# Autodesk Inventor assembly: 000 Ensamblaje hw_LM - BASIC
(part 2 of 4)
575. UND_0201CR___ _________:138
576. UND_0201CR___ _________:139 — Flush:890
577. UND_0201CR___ _________:140
578. UND_0201CR___ _________:141
579. UND_0201CR___ _________:142
580. UND_0201CR___ _________:143
581. UND_0201CR___ _________:144 — Flush:891, Flush:918
582. UND_0201CR___ _________:145
583. UND_0201CR___ _________:146 — Flush:920
584. UND_0201CR___ _________:147
585. UND_0201CR___ _________:148 — Flush:891
586. UND_0201CR___ _________:149 — Flush:889
587. UND_0201CR___ _________:150
588. UND_0201CR___ _________:151
589. UND_0201CR___ _________:152
590. UND_0201CR___ _________:153
591. UND_0201CR___ _________:154
592. UND_0201CR___ _________:155
593. UND_0201CR___ _________:156
594. UND_0201CR___ _________:157
595. UND_0201CR___ _________:158
596. UND_0201CR___ _________:159 — Flush:918, Flush:919
597. UND_0201CR___ _________:160
598. UND_0201CR___ _________:161
599. UND_0201CR___ _________:162 — Flush:921
600. UND_0201CR___ _________:163
601. UND_0201CR___ _________:164
602. UND_0201CR___ _________:165 — Flush:1036, Flush:1136
603. UND_0201CR___ _________:166
604. UND_0201CR___ _________:167 — Flush:920, Flush:949, Flush:973
605. UND_0201CR___ _________:168 — Flush:919
606. UND_0201CR___ _________:169
607. UND_0201CR___ _________:170 — Flush:953
608. UND_0201CR___ _________:171 — Flush:921, Flush:952
609. UND_0201CR___ _________:172
610. UND_0201CR___ _________:173
611. UND_0201CR___ _________:174
612. UND_0201CR___ _________:175 — Flush:950
613. UND_0201CR___ _________:176 — Flush:948, Flush:949
614. UND_0201CR___ _________:177
615. UND_0201CR___ _________:178 — Flush:952, Flush:974, Flush:998
616. UND_0201CR___ _________:179
617. UND_0201CR___ _________:180 — Flush:951
618. UND_0201CR___ _________:181
619. UND_0201CR___ _________:182 — Flush:953, Flush:976
620. UND_0201CR___ _________:183
621. UND_0201CR___ _________:184
622. UND_0201CR___ _________:185 — Flush:948
623. UND_0201CR___ _________:186
624. UND_0201CR___ _________:187 — Flush:951
625. UND_0201CR___ _________:188
626. UND_0201CR___ _________:189
627. UND_0201CR___ _________:190
628. UND_0201CR___ _________:191 — Flush:950
629. UND_0201CR___ _________:192
630. UND_0201CR___ _________:193 — Flush:973, Flush:976
631. UND_0201CR___ _________:194 — Flush:974
632. UND_0201CR___ _________:195 — Flush:975
633. UND_0201CR___ _________:196
634. UND_0201CR___ _________:197
635. UND_0201CR___ _________:198 — Flush:997
636. UND_0201CR___ _________:199
637. UND_0201CR___ _________:200
638. UND_0201CR___ _________:201 — Flush:996
639. UND_0201CR___ _________:202 — Flush:975
640. UND_0201CR___ _________:203
641. UND_0201CR___ _________:204
642. UND_0201CR___ _________:205
643. UND_0201CR___ _________:206
644. UND_0201CR___ _________:207 — Flush:997
645. UND_0201CR___ _________:208 — Flush:1009
646. UND_0201CR___ _________:209
647. UND_0201CR___ _________:210
648. UND_0201CR___ _________:211
649. UND_0201CR___ _________:212
650. UND_0201CR___ _________:213 — Flush:996
651. UND_0201CR___ _________:214
652. UND_0201CR___ _________:215
653. UND_0201CR___ _________:216
654. UND_0201CR___ _________:217
655. UND_0201CR___ _________:218 — Flush:998
656. UND_0201CR___ _________:219
657. UND_0201CR___ _________:220 — Flush:1008
658. UND_0201CR___ _________:221 — Flush:1008, Flush:1031
659. UND_0201CR___ _________:222
660. UND_0201CR___ _________:223 — Flush:1009
661. UND_0201CR___ _________:224
662. UND_0201CR___ _________:225 — Flush:1032
663. UND_0201CR___ _________:226 — Flush:1029
664. UND_0201CR___ _________:227
665. UND_0201CR___ _________:228
666. UND_0201CR___ _________:229 — Flush:1029, Flush:1069
667. UND_0201CR___ _________:230 — Flush:1033
668. UND_0201CR___ _________:231 — Flush:1034
669. UND_0201CR___ _________:232 — Flush:1030
670. UND_0201CR___ _________:233 — Flush:1031
671. UND_0201CR___ _________:234
672. UND_0201CR___ _________:235
673. UND_0201CR___ _________:236 — Flush:1028, Flush:1036
674. UND_0201CR___ _________:237 — Flush:1033, Flush:1035
675. UND_0201CR___ _________:238 — Flush:1028
676. UND_0201CR___ _________:239
677. UND_0201CR___ _________:240 — Flush:1030, Flush:1034
678. UND_0201CR___ _________:241
679. UND_0201CR___ _________:242 — Flush:1032
680. UND_0201CR___ _________:243
681. UND_0201CR___ _________:244
682. UND_0201CR___ _________:249
683. UND_0201CR___ _________:250
684. UND_0201CR___ _________:251
685. UND_0201CR___ _________:252
686. UND_0201CR___ _________:253
687. UND_0201CR___ _________:257
688. UND_0201CR___ _________:261
689. UND_0201CR___ _________:262
690. UND_0201CR___ _________:266 — Flush:1069
691. UND_0201CR___ _________:267
692. UND_0201CR___ _________:268
693. UND_0201CR___ _________:269 — Flush:1130
694. UND_0201CR___ _________:270 — Flush:1135
695. UND_0201CR___ _________:271 — Flush:1135, Flush:1136
## Relationships (1031: Flush 748, Angle 167, Mate 116)
- Mate:1: hw_LM - PCB:1
- Flush:1: hw_LM - PCB:1
- Flush:2: hw_LM - PCB:1
- Mate:33: hw_LM - PCB:1 ↔ Sen-Z-f:1
- Mate:35: hw_LM - PCB:1 ↔ Sen-XY-f:1
- Flush:16: Sen-XY-f:1 ↔ Sen-XY-f:2
- Mate:60: hw_LM - PCB:1 ↔ MAGI2C:1
- Mate:72: hw_LM - PCB:1 ↔ RES-1.6K_1%_0402:1
- [Flush]: RES-1.6K_1%_0402:9 ↔ RES-1.6K_1%_0402:8
- Flush:59: RES-1.6K_1%_0402:9 ↔ RES-1.6K_1%_0402:8
- Flush:64: RES-1.6K_1%_0402:14 ↔ RES-1.6K_1%_0402:16
- Flush:65: RES-1.6K_1%_0402:14 ↔ RES-1.6K_1%_0402:15
- Flush:66: RES-1.6K_1%_0402:13 ↔ RES-1.6K_1%_0402:15
- [Flush]: RES-1.6K_1%_0402:18 ↔ RES-1.6K_1%_0402:20
- Flush:73: RES-1.6K_1%_0402:16 ↔ RES-1.6K_1%_0402:18
- [Flush]: RES-1.6K_1%_0402:22 ↔ RES-1.6K_1%_0402:25
- [Flush]: RES-1.6K_1%_0402:27 ↔ RES-1.6K_1%_0402:28
- [Flush]: RES-1.6K_1%_0402:27 ↔ RES-1.6K_1%_0402:28
- Flush:85: RES-1.6K_1%_0402:22 ↔ RES-1.6K_1%_0402:27
- Flush:86: RES-1.6K_1%_0402:22 ↔ RES-1.6K_1%_0402:29
- [Flush]: RES-1.6K_1%_0402:34 ↔ RES-1.6K_1%_0402:35
- [Flush]: RES-1.6K_1%_0402:40 ↔ RES-1.6K_1%_0402:42
- Flush:118: RES-1.6K_1%_0402:16 ↔ RES-1.6K_1%_0402:40
- Flush:138: RES-1.6K_1%_0402:44 ↔ RES-1.6K_1%_0402:56
- Mate:84: hw_LM - PCB:1 ↔ RES-1.6K_1%_0402:56
- Flush:146: RES-1.6K_1%_0402:56 ↔ RES-1.6K_1%_0402:58
- Flush:151: RES-1.6K_1%_0402:56 ↔ RES-1.6K_1%_0402:59
- Flush:153: RES-1.6K_1%_0402:50 ↔ RES-1.6K_1%_0402:51
- [Flush]: RES-1.6K_1%_0402:60 ↔ RES-1.6K_1%_0402:62
- Flush:159: RES-1.6K_1%_0402:60 ↔ RES-1.6K_1%_0402:63
- Flush:160: RES-1.6K_1%_0402:61 ↔ RES-1.6K_1%_0402:63
- [Flush]: RES-1.6K_1%_0402:64 ↔ RES-1.6K_1%_0402:66
- [Flush]: RES-1.6K_1%_0402:64 ↔ RES-1.6K_1%_0402:67
- [Flush]: RES-1.6K_1%_0402:65 ↔ RES-1.6K_1%_0402:67
- Flush:164: RES-1.6K_1%_0402:62 ↔ RES-1.6K_1%_0402:65
- [Flush]: RES-1.6K_1%_0402:69 ↔ RES-1.6K_1%_0402:71
- Flush:168: RES-1.6K_1%_0402:62 ↔ RES-1.6K_1%_0402:69
- [Flush]: RES-1.6K_1%_0402:72 ↔ RES-1.6K_1%_0402:73
- [Flush]: RES-1.6K_1%_0402:72 ↔ RES-1.6K_1%_0402:73
- Flush:174: RES-1.6K_1%_0402:72 ↔ RES-1.6K_1%_0402:75
- [Flush]: RES-1.6K_1%_0402:76 ↔ RES-1.6K_1%_0402:77
- [Flush]: RES-1.6K_1%_0402:76 ↔ RES-1.6K_1%_0402:77
- [Flush]: RES-1.6K_1%_0402:78 ↔ RES-1.6K_1%_0402:79
- [Flush]: RES-1.6K_1%_0402:78 ↔ RES-1.6K_1%_0402:79
- [Flush]: RES-1.6K_1%_0402:77 ↔ RES-1.6K_1%_0402:78
- [Flush]: RES-1.6K_1%_0402:76 ↔ RES-1.6K_1%_0402:79
- Flush:182: RES-1.6K_1%_0402:67 ↔ RES-1.6K_1%_0402:79
- Flush:183: RES-1.6K_1%_0402:66 ↔ RES-1.6K_1%_0402:76
- [Flush]: RES-1.6K_1%_0402:80 ↔ RES-1.6K_1%_0402:81
- [Flush]: RES-1.6K_1%_0402:80 ↔ RES-1.6K_1%_0402:81
- Flush:186: RES-1.6K_1%_0402:78 ↔ RES-1.6K_1%_0402:80
- [Flush]: RES-1.6K_1%_0402:84 ↔ RES-1.6K_1%_0402:85
- Flush:192: RES-1.6K_1%_0402:84 ↔ RES-1.6K_1%_0402:85
- Flush:194: RES-1.6K_1%_0402:85 ↔ RES-1.6K_1%_0402:86
- Mate:94: hw_LM - PCB:1 ↔ S32E288ABCAAMJGT:1
- Mate:95: hw_LM - PCB:1 ↔ DP83867ERGZT:1
- Mate:107: hw_LM - PCB:1 ↔ SML-D12V8WT86C:2
- Mate:108: hw_LM - PCB:1 ↔ SML-D12V8WT86C:3
- Mate:109: hw_LM - PCB:1 ↔ SML-D12V8WT86C:4
- Mate:110: hw_LM - PCB:1 ↔ SML-D12V8WT86C:5
- Mate:112: hw_LM - PCB:1 ↔ RES-1.6K_1%_0402:92
- Mate:113: hw_LM - PCB:1 ↔ RES-1.6K_1%_0402:91
- Mate:114: hw_LM - PCB:1 ↔ RES-1.6K_1%_0402:90
- Mate:115: hw_LM - PCB:1 ↔ RES-1.6K_1%_0402:89
- Flush:202: SML-D12V8WT86C:2 ↔ SML-D12V8WT86C:6
- Flush:204: RES-1.6K_1%_0402:89 ↔ RES-1.6K_1%_0402:94
- Flush:205: RES-1.6K_1%_0402:89 ↔ RES-1.6K_1%_0402:90
- Flush:206: RES-1.6K_1%_0402:90 ↔ RES-1.6K_1%_0402:91
- Flush:207: RES-1.6K_1%_0402:91 ↔ RES-1.6K_1%_0402:92
- Mate:116: hw_LM - PCB:1 ↔ SMA6J64CA:1
- Mate:117: hw_LM - PCB:1 ↔ SMA6J64CA:2
- Mate:118: hw_LM - PCB:1 ↔ C1210C472KGRACAUTO:1
- Mate:123: hw_LM - PCB:1 ↔ 1812CAN-113NRC:1
- Mate:124: hw_LM - PCB:1 ↔ TCAN1462VDRBRQ1:5
- Flush:228: C1210C472KGRACAUTO:11 ↔ C1210C472KGRACAUTO:12
- Flush:230: C1210C472KGRACAUTO:11 ↔ C1210C472KGRACAUTO:12
- Flush:232: C1210C472KGRACAUTO:11 ↔ C1210C472KGRACAUTO:12
- [Flush]: RES-1.6K_1%_0402:108 ↔ RES-1.6K_1%_0402:109
- Flush:249: RES-1.6K_1%_0402:107 ↔ RES-1.6K_1%_0402:109
- Flush:251: RES-1.6K_1%_0402:104 ↔ RES-1.6K_1%_0402:109
- Flush:252: RES-1.6K_1%_0402:105 ↔ RES-1.6K_1%_0402:107
- [Flush]: RES-1.6K_1%_0402:114 ↔ RES-1.6K_1%_0402:115
- [Flush]: RES-1.6K_1%_0402:113 ↔ RES-1.6K_1%_0402:115
- [Flush]: RES-1.6K_1%_0402:110 ↔ RES-1.6K_1%_0402:115
- Flush:261: RES-1.6K_1%_0402:105 ↔ RES-1.6K_1%_0402:113
- [Flush]: RES-1.6K_1%_0402:117 ↔ RES-1.6K_1%_0402:118
- [Flush]: RES-1.6K_1%_0402:120 ↔ RES-1.6K_1%_0402:121
- [Flush]: RES-1.6K_1%_0402:118 ↔ RES-1.6K_1%_0402:120
- [Flush]: RES-1.6K_1%_0402:123 ↔ RES-1.6K_1%_0402:124
- Flush:278: RES-1.6K_1%_0402:105 ↔ RES-1.6K_1%_0402:120
- [Flush]: RES-1.6K_1%_0402:129 ↔ RES-1.6K_1%_0402:130
- [Flush]: RES-1.6K_1%_0402:132 ↔ RES-1.6K_1%_0402:133
- [Flush]: RES-1.6K_1%_0402:131 ↔ RES-1.6K_1%_0402:133
- [Flush]: RES-1.6K_1%_0402:130 ↔ RES-1.6K_1%_0402:132
- [Flush]: RES-1.6K_1%_0402:128 ↔ RES-1.6K_1%_0402:133
- [Flush]: RES-1.6K_1%_0402:129 ↔ RES-1.6K_1%_0402:131
- [Flush]: RES-1.6K_1%_0402:135 ↔ RES-1.6K_1%_0402:136
- [Flush]: RES-1.6K_1%_0402:138 ↔ RES-1.6K_1%_0402:139
- [Flush]: RES-1.6K_1%_0402:137 ↔ RES-1.6K_1%_0402:139
- [Flush]: RES-1.6K_1%_0402:136 ↔ RES-1.6K_1%_0402:138
- [Flush]: RES-1.6K_1%_0402:134 ↔ RES-1.6K_1%_0402:139
- [Flush]: RES-1.6K_1%_0402:135 ↔ RES-1.6K_1%_0402:137
- [Flush]: RES-1.6K_1%_0402:131 ↔ RES-1.6K_1%_0402:136
- [Flush]: RES-1.6K_1%_0402:129 ↔ RES-1.6K_1%_0402:137
- [Flush]: RES-1.6K_1%_0402:132 ↔ RES-1.6K_1%_0402:138
- Flush:294: RES-1.6K_1%_0402:134 ↔ RES-1.6K_1%_0402:139
- Flush:295: RES-1.6K_1%_0402:117 ↔ RES-1.6K_1%_0402:139
- Flush:296: RES-1.6K_1%_0402:113 ↔ RES-1.6K_1%_0402:137
- [Flush]: RES-1.6K_1%_0402:140 ↔ RES-1.6K_1%_0402:141
- [Flush]: RES-1.6K_1%_0402:144 ↔ RES-1.6K_1%_0402:145
- [Flush]: RES-1.6K_1%_0402:143 ↔ RES-1.6K_1%_0402:145
- [Flush]: RES-1.6K_1%_0402:142 ↔ RES-1.6K_1%_0402:145
- [Flush]: RES-1.6K_1%_0402:148 ↔ RES-1.6K_1%_0402:149
- [Flush]: RES-1.6K_1%_0402:147 ↔ RES-1.6K_1%_0402:149
- [Flush]: RES-1.6K_1%_0402:146 ↔ RES-1.6K_1%_0402:149
- [Flush]: RES-1.6K_1%_0402:144 ↔ RES-1.6K_1%_0402:148
- [Flush]: RES-1.6K_1%_0402:146 ↔ RES-1.6K_1%_0402:149
- [Flush]: RES-1.6K_1%_0402:140 ↔ RES-1.6K_1%_0402:149
- [Flush]: RES-1.6K_1%_0402:150 ↔ RES-1.6K_1%_0402:151
- [Flush]: RES-1.6K_1%_0402:158 ↔ RES-1.6K_1%_0402:159
- [Flush]: RES-1.6K_1%_0402:157 ↔ RES-1.6K_1%_0402:159
- [Flush]: RES-1.6K_1%_0402:156 ↔ RES-1.6K_1%_0402:159
- [Flush]: RES-1.6K_1%_0402:156 ↔ RES-1.6K_1%_0402:159
- [Flush]: RES-1.6K_1%_0402:150 ↔ RES-1.6K_1%_0402:159
- Flush:317: RES-1.6K_1%_0402:145 ↔ RES-1.6K_1%_0402:157
- Flush:318: RES-1.6K_1%_0402:147 ↔ RES-1.6K_1%_0402:155
- Flush:319: RES-1.6K_1%_0402:113 ↔ RES-1.6K_1%_0402:150
- Flush:324: RES-1.6K_1%_0402:144 ↔ RES-1.6K_1%_0402:161
- Flush:325: RES-1.6K_1%_0402:161 ↔ RES-1.6K_1%_0402:162
- Flush:326: RES-1.6K_1%_0402:146 ↔ RES-1.6K_1%_0402:160
- Flush:327: RES-1.6K_1%_0402:143 ↔ RES-1.6K_1%_0402:164
- Flush:328: RES-1.6K_1%_0402:145 ↔ RES-1.6K_1%_0402:161
- Mate:131: hw_LM - PCB:1 ↔ LTC2875MPDD#PBF:1
- Mate:132: hw_LM - PCB:1 ↔ UQFN-16:1
- Angle:59 (0 deg): hw_LM - PCB:1 ↔ UQFN-16:1
- Flush:331: LTC2875MPDD#PBF:1 ↔ LTC2875MPDD#PBF:2
- Mate:134: hw_LM - PCB:1 ↔ TPS3897ADRYT:1
- Angle:62 (180 deg): hw_LM - PCB:1 ↔ PESD2CANFD27V-UX:1
- Mate:135: hw_LM - PCB:1 ↔ PESD2CANFD27V-UX:1
- Angle:63 (0 deg): SMA6J64CA:1 ↔ PESD2CANFD27V-UX:1
- Angle:64 (180 deg): hw_LM - PCB:1 ↔ DMN2710UTQ-7:1
- Mate:136: hw_LM - PCB:1 ↔ DMN2710UTQ-7:1
- Flush:336: C0603C103K1RECAUTO:14 ↔ C0603C103K1RECAUTO:15
- [Flush]: RES-1.6K_1%_0402:166 ↔ RES-1.6K_1%_0402:168
- Flush:346: RES-1.6K_1%_0402:146 ↔ RES-1.6K_1%_0402:168
- [Flush]: RES-1.6K_1%_0402:183 ↔ RES-1.6K_1%_0402:184
- [Flush]: RES-1.6K_1%_0402:182 ↔ RES-1.6K_1%_0402:184
- [Flush]: RES-1.6K_1%_0402:181 ↔ RES-1.6K_1%_0402:184
- [Flush]: RES-1.6K_1%_0402:178 ↔ RES-1.6K_1%_0402:183
- [Flush]: RES-1.6K_1%_0402:179 ↔ RES-1.6K_1%_0402:181
- [Flush]: RES-1.6K_1%_0402:180 ↔ RES-1.6K_1%_0402:184
- [Flush]: RES-1.6K_1%_0402:178 ↔ RES-1.6K_1%_0402:184
- [Flush]: RES-1.6K_1%_0402:179 ↔ RES-1.6K_1%_0402:185
- [Flush]: RES-1.6K_1%_0402:191 ↔ RES-1.6K_1%_0402:192
- [Flush]: RES-1.6K_1%_0402:190 ↔ RES-1.6K_1%_0402:192
- [Flush]: RES-1.6K_1%_0402:189 ↔ RES-1.6K_1%_0402:192
- [Flush]: RES-1.6K_1%_0402:186 ↔ RES-1.6K_1%_0402:191
- [Flush]: RES-1.6K_1%_0402:187 ↔ RES-1.6K_1%_0402:189
- [Flush]: RES-1.6K_1%_0402:188 ↔ RES-1.6K_1%_0402:192
- [Flush]: RES-1.6K_1%_0402:186 ↔ RES-1.6K_1%_0402:192
- [Flush]: RES-1.6K_1%_0402:187 ↔ RES-1.6K_1%_0402:193
- [Flush]: RES-1.6K_1%_0402:198 ↔ RES-1.6K_1%_0402:200
- [Flush]: RES-1.6K_1%_0402:197 ↔ RES-1.6K_1%_0402:200
- [Flush]: RES-1.6K_1%_0402:195 ↔ RES-1.6K_1%_0402:197
- [Flush]: RES-1.6K_1%_0402:196 ↔ RES-1.6K_1%_0402:200
- [Flush]: RES-1.6K_1%_0402:194 ↔ RES-1.6K_1%_0402:200
- [Flush]: RES-1.6K_1%_0402:195 ↔ RES-1.6K_1%_0402:201
- Flush:382: RES-1.6K_1%_0402:170 ↔ RES-1.6K_1%_0402:183
- Flush:383: RES-1.6K_1%_0402:183 ↔ RES-1.6K_1%_0402:198
- Flush:384: RES-1.6K_1%_0402:185 ↔ RES-1.6K_1%_0402:200
- Flush:386: RES-1.6K_1%_0402:187 ↔ RES-1.6K_1%_0402:197
- Flush:387: RES-1.6K_1%_0402:188 ↔ RES-1.6K_1%_0402:201
- Flush:388: RES-1.6K_1%_0402:189 ↔ RES-1.6K_1%_0402:200
- Angle:69 (0 deg): RES-1.6K_1%_0402:191 ↔ RES-1.6K_1%_0402:192
- Angle:70 (0 deg): RES-1.6K_1%_0402:190 ↔ RES-1.6K_1%_0402:191
- Angle:71 (0 deg): RES-1.6K_1%_0402:189 ↔ RES-1.6K_1%_0402:190
- Angle:72 (0 deg): RES-1.6K_1%_0402:189 ↔ RES-1.6K_1%_0402:193
- Angle:73 (0 deg): RES-1.6K_1%_0402:186 ↔ RES-1.6K_1%_0402:193
- Angle:74 (0 deg): RES-1.6K_1%_0402:186 ↔ RES-1.6K_1%_0402:187
- Angle:75 (0 deg): RES-1.6K_1%_0402:188 ↔ RES-1.6K_1%_0402:189
- [Flush]: RES-1.6K_1%_0402:207 ↔ RES-1.6K_1%_0402:208
- [Flush]: RES-1.6K_1%_0402:202 ↔ RES-1.6K_1%_0402:207
- [Flush]: RES-1.6K_1%_0402:202 ↔ RES-1.6K_1%_0402:208
- [Flush]: RES-1.6K_1%_0402:203 ↔ RES-1.6K_1%_0402:209
- [Angle] (0 deg): RES-1.6K_1%_0402:207 ↔ RES-1.6K_1%_0402:208
- [Angle] (0 deg): RES-1.6K_1%_0402:202 ↔ RES-1.6K_1%_0402:209
- [Angle] (0 deg): RES-1.6K_1%_0402:202 ↔ RES-1.6K_1%_0402:203
- Flush:398: RES-1.6K_1%_0402:191 ↔ RES-1.6K_1%_0402:202
- [Flush]: RES-1.6K_1%_0402:212 ↔ RES-1.6K_1%_0402:213
- [Flush]: RES-1.6K_1%_0402:212 ↔ RES-1.6K_1%_0402:213
- [Flush]: RES-1.6K_1%_0402:211 ↔ RES-1.6K_1%_0402:213
- [Flush]: RES-1.6K_1%_0402:211 ↔ RES-1.6K_1%_0402:213
- [Flush]: RES-1.6K_1%_0402:215 ↔ RES-1.6K_1%_0402:216
- [Flush]: RES-1.6K_1%_0402:214 ↔ RES-1.6K_1%_0402:216
- Flush:417: RES-1.6K_1%_0402:215 ↔ RES-1.6K_1%_0402:221
- Flush:423: DMN2710UTQ-7:7 ↔ DMN2710UTQ-7:8
- Mate:139: hw_LM - PCB:1 ↔ RES-1.6K_1%_0402:97
- Mate:153: hw_LM - PCB:1 ↔ TPD4E05U06QDQARQ1:1
- Flush:447: TPD4E05U06QDQARQ1:1 ↔ TPD4E05U06QDQARQ1:3
- Flush:448: TPD4E05U06QDQARQ1:2 ↔ TPD4E05U06QDQARQ1:3
- Mate:154: hw_LM - PCB:1 ↔ P3767-pcba-envelop_20230310-modificada:1
- Mate:155: hw_LM - PCB:1 ↔ P3767-pcba-envelop_20230310-modificada:1
- Flush:450: RES-1.6K_1%_0402:226 ↔ RES-1.6K_1%_0402:227
- Flush:451: RES-1.6K_1%_0402:97 ↔ RES-1.6K_1%_0402:226
- Flush:452: RES-1.6K_1%_0402:224 ↔ RES-1.6K_1%_0402:226
- Flush:453: RES-1.6K_1%_0402:225 ↔ RES-1.6K_1%_0402:226
- Flush:454: RES-1.6K_1%_0402:225 ↔ RES-1.6K_1%_0402:227
- [Flush]: RES-1.6K_1%_0402:234 ↔ RES-1.6K_1%_0402:235
- [Flush]: RES-1.6K_1%_0402:232 ↔ RES-1.6K_1%_0402:234
- [Flush]: RES-1.6K_1%_0402:233 ↔ RES-1.6K_1%_0402:234
- [Flush]: RES-1.6K_1%_0402:233 ↔ RES-1.6K_1%_0402:235
- Flush:465: RES-1.6K_1%_0402:228 ↔ RES-1.6K_1%_0402:233
- Flush:466: RES-1.6K_1%_0402:224 ↔ RES-1.6K_1%_0402:235
- Flush:467: RES-1.6K_1%_0402:97 ↔ RES-1.6K_1%_0402:226
- [Flush]: RES-1.6K_1%_0402:238 ↔ RES-1.6K_1%_0402:239
- [Flush]: RES-1.6K_1%_0402:236 ↔ RES-1.6K_1%_0402:238
- [Flush]: RES-1.6K_1%_0402:237 ↔ RES-1.6K_1%_0402:238
- [Flush]: RES-1.6K_1%_0402:237 ↔ RES-1.6K_1%_0402:239
- [Flush]: RES-1.6K_1%_0402:242 ↔ RES-1.6K_1%_0402:243
- [Flush]: RES-1.6K_1%_0402:240 ↔ RES-1.6K_1%_0402:242
- [Flush]: RES-1.6K_1%_0402:241 ↔ RES-1.6K_1%_0402:242
- [Flush]: RES-1.6K_1%_0402:241 ↔ RES-1.6K_1%_0402:243
- Flush:476: RES-1.6K_1%_0402:226 ↔ RES-1.6K_1%_0402:239
- Flush:477: RES-1.6K_1%_0402:232 ↔ RES-1.6K_1%_0402:237
- Flush:478: RES-1.6K_1%_0402:236 ↔ RES-1.6K_1%_0402:241
- Flush:479: RES-1.6K_1%_0402:97 ↔ RES-1.6K_1%_0402:234
- Flush:480: RES-1.6K_1%_0402:234 ↔ RES-1.6K_1%_0402:240
- [Flush]: RES-1.6K_1%_0402:245 ↔ RES-1.6K_1%_0402:247
- [Flush]: RES-1.6K_1%_0402:249 ↔ RES-1.6K_1%_0402:251
- Flush:491: RES-1.6K_1%_0402:247 ↔ RES-1.6K_1%_0402:249
- Flush:492: RES-1.6K_1%_0402:97 ↔ RES-1.6K_1%_0402:249
- [Flush]: RES-1.6K_1%_0402:258 ↔ RES-1.6K_1%_0402:259
- [Flush]: RES-1.6K_1%_0402:256 ↔ RES-1.6K_1%_0402:258
- [Flush]: RES-1.6K_1%_0402:257 ↔ RES-1.6K_1%_0402:258
- [Flush]: RES-1.6K_1%_0402:257 ↔ RES-1.6K_1%_0402:259
- Flush:502: RES-1.6K_1%_0402:253 ↔ RES-1.6K_1%_0402:259
- Flush:503: RES-1.6K_1%_0402:248 ↔ RES-1.6K_1%_0402:258
- Flush:504: RES-1.6K_1%_0402:253 ↔ RES-1.6K_1%_0402:256
- [Flush]: RES-1.6K_1%_0402:261 ↔ RES-1.6K_1%_0402:262
- [Flush]: RES-1.6K_1%_0402:260 ↔ RES-1.6K_1%_0402:261
- [Flush]: RES-1.6K_1%_0402:260 ↔ RES-1.6K_1%_0402:262
- [Flush]: RES-1.6K_1%_0402:264 ↔ RES-1.6K_1%_0402:265
- [Flush]: RES-1.6K_1%_0402:263 ↔ RES-1.6K_1%_0402:264
- [Flush]: RES-1.6K_1%_0402:263 ↔ RES-1.6K_1%_0402:265
- Angle:91 (0 deg): hw_LM - PCB:1 ↔ RES-1.6K_1%_0402:258
- Angle:92 (0 deg): RES-1.6K_1%_0402:258 ↔ RES-1.6K_1%_0402:259
- Angle:93 (0 deg): RES-1.6K_1%_0402:257 ↔ RES-1.6K_1%_0402:258
- Angle:94 (0 deg): RES-1.6K_1%_0402:257 ↔ RES-1.6K_1%_0402:264
- Angle:95 (0 deg): RES-1.6K_1%_0402:263 ↔ RES-1.6K_1%_0402:264
- Angle:96 (0 deg): RES-1.6K_1%_0402:264 ↔ RES-1.6K_1%_0402:265
- Angle:97 (0 deg): RES-1.6K_1%_0402:257 ↔ RES-1.6K_1%_0402:260
- Angle:98 (0 deg): RES-1.6K_1%_0402:260 ↔ RES-1.6K_1%_0402:261
- Angle:99 (0 deg): RES-1.6K_1%_0402:260 ↔ RES-1.6K_1%_0402:262
- [Flush]: RES-1.6K_1%_0402:266 ↔ RES-1.6K_1%_0402:267
- [Flush]: RES-1.6K_1%_0402:269 ↔ RES-1.6K_1%_0402:270
- [Flush]: RES-1.6K_1%_0402:268 ↔ RES-1.6K_1%_0402:269
- [Flush]: RES-1.6K_1%_0402:268 ↔ RES-1.6K_1%_0402:270
- [Angle] (0 deg): RES-1.6K_1%_0402:266 ↔ RES-1.6K_1%_0402:267
- [Angle] (0 deg): RES-1.6K_1%_0402:268 ↔ RES-1.6K_1%_0402:269
- [Angle] (0 deg): RES-1.6K_1%_0402:269 ↔ RES-1.6K_1%_0402:270
- Flush:515: RES-1.6K_1%_0402:259 ↔ RES-1.6K_1%_0402:268
- Flush:516: RES-1.6K_1%_0402:266 ↔ RES-1.6K_1%_0402:267
- Flush:517: RES-1.6K_1%_0402:263 ↔ RES-1.6K_1%_0402:267
- Flush:518: RES-1.6K_1%_0402:97 ↔ RES-1.6K_1%_0402:270
- [Flush]: RES-1.6K_1%_0402:274 ↔ RES-1.6K_1%_0402:275
- [Flush]: RES-1.6K_1%_0402:273 ↔ RES-1.6K_1%_0402:274
- [Flush]: RES-1.6K_1%_0402:273 ↔ RES-1.6K_1%_0402:275
- [Angle] (0 deg): RES-1.6K_1%_0402:273 ↔ RES-1.6K_1%_0402:274
- [Angle] (0 deg): RES-1.6K_1%_0402:274 ↔ RES-1.6K_1%_0402:275
- [Flush]: RES-1.6K_1%_0402:276 ↔ RES-1.6K_1%_0402:277
- [Flush]: RES-1.6K_1%_0402:279 ↔ RES-1.6K_1%_0402:280
- [Flush]: RES-1.6K_1%_0402:278 ↔ RES-1.6K_1%_0402:279
- [Flush]: RES-1.6K_1%_0402:278 ↔ RES-1.6K_1%_0402:280
- [Angle] (0 deg): RES-1.6K_1%_0402:276 ↔ RES-1.6K_1%_0402:277
- [Angle] (0 deg): RES-1.6K_1%_0402:278 ↔ RES-1.6K_1%_0402:279
- [Angle] (0 deg): RES-1.6K_1%_0402:279 ↔ RES-1.6K_1%_0402:280
- [Flush]: RES-1.6K_1%_0402:272 ↔ RES-1.6K_1%_0402:278
- [Flush]: RES-1.6K_1%_0402:276 ↔ RES-1.6K_1%_0402:277
- [Flush]: RES-1.6K_1%_0402:273 ↔ RES-1.6K_1%_0402:277
- Flush:530: RES-1.6K_1%_0402:277 ↔ RES-1.6K_1%_0402:278
- Flush:532: RES-1.6K_1%_0402:272 ↔ RES-1.6K_1%_0402:273
- Flush:533: RES-1.6K_1%_0402:275 ↔ RES-1.6K_1%_0402:278
- Flush:534: RES-1.6K_1%_0402:272 ↔ RES-1.6K_1%_0402:273
- Flush:535: RES-1.6K_1%_0402:263 ↔ RES-1.6K_1%_0402:268
- [Flush]: RES-1.6K_1%_0402:285 ↔ RES-1.6K_1%_0402:286
- [Flush]: RES-1.6K_1%_0402:284 ↔ RES-1.6K_1%_0402:285
- [Flush]: RES-1.6K_1%_0402:284 ↔ RES-1.6K_1%_0402:286
- [Angle] (0 deg): RES-1.6K_1%_0402:284 ↔ RES-1.6K_1%_0402:285
- [Angle] (0 deg): RES-1.6K_1%_0402:285 ↔ RES-1.6K_1%_0402:286
- [Flush]: RES-1.6K_1%_0402:288 ↔ RES-1.6K_1%_0402:289
- [Flush]: RES-1.6K_1%_0402:287 ↔ RES-1.6K_1%_0402:288
- [Flush]: RES-1.6K_1%_0402:287 ↔ RES-1.6K_1%_0402:289
- [Angle] (0 deg): RES-1.6K_1%_0402:287 ↔ RES-1.6K_1%_0402:288
- [Angle] (0 deg): RES-1.6K_1%_0402:288 ↔ RES-1.6K_1%_0402:289
- [Flush]: RES-1.6K_1%_0402:286 ↔ RES-1.6K_1%_0402:287
- Flush:545: RES-1.6K_1%_0402:283 ↔ RES-1.6K_1%_0402:286
- Flush:546: RES-1.6K_1%_0402:280 ↔ RES-1.6K_1%_0402:283
- Flush:547: RES-1.6K_1%_0402:285 ↔ RES-1.6K_1%_0402:286
- Flush:548: RES-1.6K_1%_0402:286 ↔ RES-1.6K_1%_0402:289
- Flush:549: RES-1.6K_1%_0402:282 ↔ RES-1.6K_1%_0402:287
- Flush:550: RES-1.6K_1%_0402:258 ↔ RES-1.6K_1%_0402:283
- Flush:551: RES-1.6K_1%_0402:258 ↔ RES-1.6K_1%_0402:287
- [Flush]: RES-1.6K_1%_0402:290 ↔ RES-1.6K_1%_0402:291
- [Angle] (0 deg): RES-1.6K_1%_0402:290 ↔ RES-1.6K_1%_0402:291
- [Flush]: RES-1.6K_1%_0402:294 ↔ RES-1.6K_1%_0402:295
- [Flush]: RES-1.6K_1%_0402:293 ↔ RES-1.6K_1%_0402:294
- [Flush]: RES-1.6K_1%_0402:293 ↔ RES-1.6K_1%_0402:295
- [Angle] (0 deg): RES-1.6K_1%_0402:293 ↔ RES-1.6K_1%_0402:294
- [Angle] (0 deg): RES-1.6K_1%_0402:294 ↔ RES-1.6K_1%_0402:295
- [Flush]: RES-1.6K_1%_0402:297 ↔ RES-1.6K_1%_0402:298
- [Flush]: RES-1.6K_1%_0402:296 ↔ RES-1.6K_1%_0402:297
- [Flush]: RES-1.6K_1%_0402:296 ↔ RES-1.6K_1%_0402:298
- [Angle] (0 deg): RES-1.6K_1%_0402:296 ↔ RES-1.6K_1%_0402:297
- [Angle] (0 deg): RES-1.6K_1%_0402:297 ↔ RES-1.6K_1%_0402:298
- [Flush]: RES-1.6K_1%_0402:295 ↔ RES-1.6K_1%_0402:296
- [Flush]: RES-1.6K_1%_0402:294 ↔ RES-1.6K_1%_0402:295
- [Flush]: RES-1.6K_1%_0402:295 ↔ RES-1.6K_1%_0402:298
- [Flush]: RES-1.6K_1%_0402:291 ↔ RES-1.6K_1%_0402:296
- Flush:564: RES-1.6K_1%_0402:282 ↔ RES-1.6K_1%_0402:297
- Flush:565: RES-1.6K_1%_0402:282 ↔ RES-1.6K_1%_0402:290
- Flush:566: RES-1.6K_1%_0402:289 ↔ RES-1.6K_1%_0402:291
- Flush:567: RES-1.6K_1%_0402:286 ↔ RES-1.6K_1%_0402:293
- Flush:570: RES-1.6K_1%_0402:287 ↔ RES-1.6K_1%_0402:300
- [Angle] (0 deg): RES-1.6K_1%_0402:303 ↔ RES-1.6K_1%_0402:304
- [Flush]: RES-1.6K_1%_0402:309 ↔ RES-1.6K_1%_0402:310
- [Angle] (0 deg): RES-1.6K_1%_0402:309 ↔ RES-1.6K_1%_0402:310
- [Angle] (0 deg): RES-1.6K_1%_0402:307 ↔ RES-1.6K_1%_0402:308
- [Flush]: RES-1.6K_1%_0402:303 ↔ RES-1.6K_1%_0402:310
- [Flush]: RES-1.6K_1%_0402:304 ↔ RES-1.6K_1%_0402:307
- Flush:579: RES-1.6K_1%_0402:288 ↔ RES-1.6K_1%_0402:307
- Flush:580: RES-1.6K_1%_0402:303 ↔ RES-1.6K_1%_0402:310
- [Flush]: RES-1.6K_1%_0402:313 ↔ RES-1.6K_1%_0402:314
- [Angle] (0 deg): RES-1.6K_1%_0402:313 ↔ RES-1.6K_1%_0402:314
- [Angle] (0 deg): RES-1.6K_1%_0402:311 ↔ RES-1.6K_1%_0402:312
- Flush:582: RES-1.6K_1%_0402:306 ↔ RES-1.6K_1%_0402:314
- Flush:583: RES-1.6K_1%_0402:288 ↔ RES-1.6K_1%_0402:312
- Flush:584: RES-1.6K_1%_0402:283 ↔ RES-1.6K_1%_0402:313
- Flush:585: RES-1.6K_1%_0402:306 ↔ RES-1.6K_1%_0402:311
- [Flush]: RES-1.6K_1%_0402:318 ↔ RES-1.6K_1%_0402:319
- [Angle] (0 deg): RES-1.6K_1%_0402:318 ↔ RES-1.6K_1%_0402:319
- [Angle] (0 deg): RES-1.6K_1%_0402:316 ↔ RES-1.6K_1%_0402:317
- Flush:588: RES-1.6K_1%_0402:288 ↔ RES-1.6K_1%_0402:317
- Flush:589: RES-1.6K_1%_0402:283 ↔ RES-1.6K_1%_0402:318
- Flush:590: RES-1.6K_1%_0402:306 ↔ RES-1.6K_1%_0402:321
- Mate:171: ATS-NVP-3281-C2-R0:1 ↔ P3767-pcba-envelop_20230310-modificada:1
- Flush:594: RES-1.6K_1%_0402:291 ↔ RES-1.6K_1%_0402:309
- Flush:595: RES-1.6K_1%_0402:225 ↔ RES-1.6K_1%_0402:262
- Flush:596: RES-1.6K_1%_0402:311 ↔ RES-1.6K_1%_0402:316
- Flush:597: RES-1.6K_1%_0402:312 ↔ RES-1.6K_1%_0402:315
- Flush:603: DMN2710UTQ-7:7 ↔ DMN2710UTQ-7:10
- Mate:187: hw_LM - PCB:1 ↔ LTC7103MPUHE#PBF:1
- Mate:188: hw_LM - PCB:1 ↔ XAL4020-601MEC:3
- Flush:611: SML-D12V8WT86C:2 ↔ SML-D12V8WT86C:7
- Mate:194: hw_LM - PCB:1 ↔ SARA:1
- Angle:142 (90 deg): hw_LM - PCB:1 ↔ Sen-Z-f:1
- Mate:199: hw_LM - PCB:1 ↔ 749020112B:1
- Angle:149 (0 deg): hw_LM - PCB:1 ↔ 749020112B:1
- Mate:200: hw_LM - PCB:1 ↔ 749020112B:2
- Mate:203: hw_LM - PCB:1 ↔ AQ24CANFD-02HTG:8
- Flush:614: TPD4E05U06QDQARQ1:3 ↔ TPD4E05U06QDQARQ1:4
- Flush:615: TPD4E05U06QDQARQ1:4 ↔ TPD4E05U06QDQARQ1:5
- Mate:210: hw_LM - PCB:1 ↔ SQJ402EP-T1_GE3:1
- Mate:213: hw_LM - PCB:1 ↔ TPD4E05U06QDQARQ1:6
- Mate:216: hw_LM - PCB:1 ↔ T495B107M006ATE700:3
- Flush:625: TCAN1462VDRBRQ1:5 ↔ TCAN1462VDRBRQ1:6
- Flush:627: XAL4020-601MEC:3 ↔ XAL4020-601MEC:6
- Mate:219: hw_LM - PCB:1 ↔ SQJ402EP-T1_GE3:2
- Mate:220: hw_LM - PCB:1 ↔ SQJ402EP-T1_GE3:2
- Mate:222: hw_LM - PCB:1 ↔ C1210C472KGRACAUTO:19
- Flush:629: C1210C472KGRACAUTO:12 ↔ C1210C472KGRACAUTO:20
- Flush:631: C0805X104K5RAC3316:3 ↔ C0805X104K5RAC3316:4
- Mate:224: hw_LM - PCB:1 ↔ TPS57112CQRTERQ1:1
- Mate:225: hw_LM - PCB:1 ↔ AQ05C-01FTG:3
- Mate:226: hw_LM - PCB:1 ↔ ECS-2520MVQ-250-CN-TR:1
- Mate:227: hw_LM - PCB:1 ↔ TCAN1462VDRBRQ1:7
- Flush:634 (3.3 mm): hw_LM - PCB:1 ↔ P3767-pcba-envelop_20230310-modificada:1
- Mate:229: hw_LM - PCB:1 ↔ AUAV-L10D-M25125-RR-N:2
- Mate:230: 2309409-2-1:1 ↔ hw_LM - PCB:1
- Mate:231: 2309409-2-1:1 ↔ hw_LM - PCB:1
- Mate:232: 2309409-2-1:1 ↔ hw_LM - PCB:1
- Mate:237: hw_LM - PCB:1 ↔ AU3PM-M3_86A:1
- Angle:169 (90 deg): hw_LM - PCB:1 ↔ AU3PM-M3_86A:1
- Mate:238: hw_LM - PCB:1 ↔ SQJ402EP-T1_GE3:1
- Mate:239: hw_LM - PCB:1 ↔ TPS7A5301QRGRRQ1:2
- Mate:240: hw_LM - PCB:1 ↔ U.FL-R-SMT-1:2
- Mate:241: hw_LM - PCB:1 ↔ U.FL-R-SMT-1:1
- Mate:242: hw_LM - PCB:1 ↔ u-blox ZED-F9P:1
- Flush:635: 1812CAN-113NRC:1 ↔ 1812CAN-113NRC:3
- Mate:243: hw_LM - PCB:1 ↔ IHLP2020CZER220M11:1
- Mate:245: hw_LM - PCB:1 ↔ R0805:11
- Mate:246: hw_LM - PCB:1 ↔ CLP-104-02-F-D-BE-TR:1
- Mate:247: hw_LM - PCB:1 ↔ BLM21PG220SN1D:4
- Mate:248: hw_LM - PCB:1 ↔ LM5146QRGYRQ1:1
- Angle:175 (0 deg): C0603C103K1RECAUTO:14 ↔ LM5146QRGYRQ1:1
- Angle:176 (0 deg): hw_LM - PCB:1 ↔ SQJ402EP-T1_GE3:2
- Mate:249: hw_LM - PCB:1 ↔ STPST8H100SFY:1
- Angle:177 (90 deg): hw_LM - PCB:1 ↔ STPST8H100SFY:1
- Flush:638: R0805:12 ↔ R0805:13
- Angle:178 (90 deg): hw_LM - PCB:1 ↔ SN74LVC1G08QDCKRQ1:2
- Mate:250: hw_LM - PCB:1 ↔ ESIM 638037665970:1
- Mate:251: hw_LM - PCB:1 ↔ ECS-400-8-33Q-ADS-TR:1
- Angle:179 (0 deg): hw_LM - PCB:1 ↔ ECS-400-8-33Q-ADS-TR:1
- Mate:252: hw_LM - PCB:1 ↔ TPS74501PQWDRBRQ1:1
- Flush:640: TPS74501PQWDRBRQ1:1 ↔ TPS74501PQWDRBRQ1:2
- [Flush]: RES-1.6K_1%_0402:323 ↔ RES-1.6K_1%_0402:324
- [Flush]: RES-1.6K_1%_0402:324 ↔ RES-1.6K_1%_0402:325
- [Flush]: RES-1.6K_1%_0402:325 ↔ RES-1.6K_1%_0402:326
- Mate:256: hw_LM - PCB:1 ↔ SN74LVC1G08QDCKRQ1:3
- Angle:181 (0 deg): hw_LM - PCB:1 ↔ SN74LVC1G08QDCKRQ1:3
- Angle:182 (180 deg): hw_LM - PCB:1 ↔ DMN2710UTQ-7:11
- Mate:257: hw_LM - PCB:1 ↔ DMN2710UTQ-7:11
- Mate:258: hw_LM - PCB:1 ↔ DMN2710UTQ-7:11
- Flush:646: DMN2710UTQ-7:12 ↔ DMN2710UTQ-7:13
- Angle:183 (0 deg): hw_LM - PCB:1 ↔ DMN2710UTQ-7:13
- Flush:647: DMN2710UTQ-7:11 ↔ DMN2710UTQ-7:12
- Angle:184 (0 deg): 2309409-2-1:1 ↔ DMN2710UTQ-7:12
- Mate:259: hw_LM - PCB:1 ↔ Body:1
- Flush:648: Body:1 ↔ Body:2
- Flush:650: PESD2CANFD27V-UX:1 ↔ PESD2CANFD27V-UX:4
- Mate:260: 9774027151R (M2,5x2,7):2 ↔ P3767-pcba-envelop_20230310-modificada:1
- Mate:261: 9774027151R (M2,5x2,7):2 ↔ P3767-pcba-envelop_20230310-modificada:1
- Mate:262: 9774027151R (M2,5x2,7):1 ↔ P3767-pcba-envelop_20230310-modificada:1
- Mate:263: 9774027151R (M2,5x2,7):1 ↔ P3767-pcba-envelop_20230310-modificada:1
- Mate:266: 3d_LM - chapa:1 ↔ P3767-pcba-envelop_20230310-modificada:1
- Mate:267: hw_LM - PCB:1 ↔ 9774090360R (M3x9):1
- Mate:268: hw_LM - PCB:1 ↔ 9774090360R (M3x9):1
- Flush:651: 9774090360R (M3x9):1 ↔ 9774090360R (M3x9):2
- Mate:269: hw_LM - PCB:1 ↔ 9774090360R (M3x9):2
- Mate:270: hw_LM - PCB:1 ↔ 9774090360R (M3x9):3
- Flush:652: T495B107M006ATE700:3 ↔ T495B107M006ATE700:5
- Angle:185 (0 deg): hw_LM - PCB:1 ↔ SOT-363-6_2P2X1P35_ONS:1
- Mate:271: hw_LM - PCB:1 ↔ SOT-363-6_2P2X1P35_ONS:1
- Angle:186 (0 deg): u-blox ZED-F9P:1 ↔ SOT-363-6_2P2X1P35_ONS:1
- Mate:272: hw_LM - PCB:1 ↔ 9774090360R (M3x9):3
- Mate:273: hw_LM - PCB:1 ↔ C1210C472KGRACAUTO:21
- Mate:274: hw_LM - PCB:1 ↔ C1210C472KGRACAUTO:22
- Angle:188 (0 deg): C1210C472KGRACAUTO:21 ↔ C1210C472KGRACAUTO:22
- Angle:189 (0 deg): hw_LM - PCB:1 ↔ BLM21PG220SN1D:4
- Angle:191 (0 deg): R0805:12 ↔ R0805:13
- Mate:275: hw_LM - PCB:1 ↔ T495B107M006ATE700:6
- Mate:276: hw_LM - PCB:1 ↔ BMI088:1
- Angle:193 (0 deg): hw_LM - PCB:1 ↔ BMI088:1
- Flush:653: C0603C103K1RECAUTO:15 ↔ C0603C103K1RECAUTO:29
- Mate:277: hw_LM - PCB:1 ↔ C1206C152KGRACAUTO:9
- Mate:278: hw_LM - PCB:1 ↔ Body:4
- Flush:656: DMN2710UTQ-7:12 ↔ DMN2710UTQ-7:14
- Angle:194 (0 deg): hw_LM - PCB:1 ↔ DMN2710UTQ-7:14
- Mate:279: hw_LM - PCB:1 ↔ AQ05C-01FTG:4
- Mate:280: hw_LM - PCB:1 ↔ AQ05C-01FTG:4
- Flush:659: C0603C103K1RECAUTO:29 ↔ C0603C103K1RECAUTO:33
- Mate:281: hw_LM - PCB:1 ↔ IAM-20680HT:1
- Mate:282: hw_LM - PCB:1 ↔ ASM330LHBG1TR:1
- Angle:195 (0 deg): hw_LM - PCB:1 ↔ T495B107M006ATE700:3
- Mate:283: 3d_LM - chapa:1 ↔ P3767-pcba-envelop_20230310-modificada:1
- Mate:284: 3d_LM - chapa:1 ↔ P3767-pcba-envelop_20230310-modificada:1
- Angle:197 (0 deg): C0805X104K5RAC3316:3 ↔ U.FL-R-SMT-1:2
- Angle:198 (180 deg): hw_LM - PCB:1 ↔ AQ24CANFD-02HTG:8
- Flush:669: RES-1.6K_1%_0402:233 ↔ RES-1.6K_1%_0402:327
- Flush:670: RES-1.6K_1%_0402:327 ↔ RES-1.6K_1%_0402:328
- Flush:671: IAM-20680HT:1 ↔ IAM-20680HT:2
- [Flush]: RES-1.6K_1%_0402:329 ↔ RES-1.6K_1%_0402:330
- [Flush]: RES-1.6K_1%_0402:329 ↔ RES-1.6K_1%_0402:330
- Flush:674: RES-1.6K_1%_0402:329 ↔ RES-1.6K_1%_0402:331
- Flush:675: RES-1.6K_1%_0402:330 ↔ RES-1.6K_1%_0402:331
- Flush:676: RES-1.6K_1%_0402:35 ↔ RES-1.6K_1%_0402:329
- Mate:285: hw_LM - PCB:1 ↔ R0805:14
- Mate:286: hw_LM - PCB:1 ↔ C0603C103K1RECAUTO:42
- Flush:678: C0603C103K1RECAUTO:42 ↔ C0603C103K1RECAUTO:44
- Angle:199 (0 deg): RES-1.6K_1%_0402:84 ↔ RES-1.6K_1%_0402:195
- Angle:200 (0 deg): SARA:1 ↔ RES-1.6K_1%_0402:195
- Mate:287: hw_LM - PCB:1 ↔ UND_0201CR___ _________:3
- Flush:679: UND_0201CR___ _________:5 ↔ UND_0201CR___ _________:8
- Flush:680: UND_0201CR___ _________:7 ↔ UND_0201CR___ _________:8
- Flush:681: UND_0201CR___ _________:4 ↔ UND_0201CR___ _________:8
- Flush:682: UND_0201CR___ _________:6 ↔ UND_0201CR___ _________:9
- Flush:683: UND_0201CR___ _________:5 ↔ UND_0201CR___ _________:6
- [Flush]: UND_0201CR___ _________:11 ↔ UND_0201CR___ _________:14
- [Flush]: UND_0201CR___ _________:13 ↔ UND_0201CR___ _________:14
- [Flush]: UND_0201CR___ _________:10 ↔ UND_0201CR___ _________:14
- [Flush]: UND_0201CR___ _________:12 ↔ UND_0201CR___ _________:15
- [Flush]: UND_0201CR___ _________:11 ↔ UND_0201CR___ _________:12
- Flush:689: UND_0201CR___ _________:9 ↔ UND_0201CR___ _________:11
- Flush:690: UND_0201CR___ _________:3 ↔ UND_0201CR___ _________:9
- Flush:691: UND_0201CR___ _________:7 ↔ UND_0201CR___ _________:10
- Flush:692: UND_0201CR___ _________:8 ↔ UND_0201CR___ _________:11
- [Flush]: UND_0201CR___ _________:17 ↔ UND_0201CR___ _________:20
- [Flush]: UND_0201CR___ _________:19 ↔ UND_0201CR___ _________:20
- [Flush]: UND_0201CR___ _________:16 ↔ UND_0201CR___ _________:20
- [Flush]: UND_0201CR___ _________:18 ↔ UND_0201CR___ _________:21
- [Flush]: UND_0201CR___ _________:17 ↔ UND_0201CR___ _________:18
- [Flush]: UND_0201CR___ _________:23 ↔ UND_0201CR___ _________:26
- [Flush]: UND_0201CR___ _________:25 ↔ UND_0201CR___ _________:26
- [Flush]: UND_0201CR___ _________:22 ↔ UND_0201CR___ _________:26
- [Flush]: UND_0201CR___ _________:24 ↔ UND_0201CR___ _________:27
- [Flush]: UND_0201CR___ _________:23 ↔ UND_0201CR___ _________:24
- [Flush]: UND_0201CR___ _________:21 ↔ UND_0201CR___ _________:23
- [Flush]: UND_0201CR___ _________:19 ↔ UND_0201CR___ _________:22
- [Flush]: UND_0201CR___ _________:20 ↔ UND_0201CR___ _________:23
- Flush:706: UND_0201CR___ _________:8 ↔ UND_0201CR___ _________:20
- Flush:707: UND_0201CR___ _________:15 ↔ UND_0201CR___ _________:18
- Flush:708: UND_0201CR___ _________:10 ↔ UND_0201CR___ _________:25
- Flush:709: UND_0201CR___ _________:3 ↔ UND_0201CR___ _________:19
- [Flush]: UND_0201CR___ _________:29 ↔ UND_0201CR___ _________:32
- [Flush]: UND_0201CR___ _________:31 ↔ UND_0201CR___ _________:32
- [Flush]: UND_0201CR___ _________:28 ↔ UND_0201CR___ _________:32
- [Flush]: UND_0201CR___ _________:30 ↔ UND_0201CR___ _________:33
- [Flush]: UND_0201CR___ _________:29 ↔ UND_0201CR___ _________:30
- [Flush]: UND_0201CR___ _________:35 ↔ UND_0201CR___ _________:38
- [Flush]: UND_0201CR___ _________:37 ↔ UND_0201CR___ _________:38
- [Flush]: UND_0201CR___ _________:34 ↔ UND_0201CR___ _________:38
- [Flush]: UND_0201CR___ _________:36 ↔ UND_0201CR___ _________:39
- [Flush]: UND_0201CR___ _________:35 ↔ UND_0201CR___ _________:36
- [Flush]: UND_0201CR___ _________:33 ↔ UND_0201CR___ _________:35
- [Flush]: UND_0201CR___ _________:31 ↔ UND_0201CR___ _________:34
- [Flush]: UND_0201CR___ _________:32 ↔ UND_0201CR___ _________:35
- [Flush]: UND_0201CR___ _________:41 ↔ UND_0201CR___ _________:44
- [Flush]: UND_0201CR___ _________:43 ↔ UND_0201CR___ _________:44
- [Flush]: UND_0201CR___ _________:40 ↔ UND_0201CR___ _________:44
- [Flush]: UND_0201CR___ _________:42 ↔ UND_0201CR___ _________:45
- [Flush]: UND_0201CR___ _________:41 ↔ UND_0201CR___ _________:42
- [Flush]: UND_0201CR___ _________:47 ↔ UND_0201CR___ _________:49
- [Flush]: UND_0201CR___ _________:48 ↔ UND_0201CR___ _________:49
- [Flush]: UND_0201CR___ _________:46 ↔ UND_0201CR___ _________:49
- [Flush]: UND_0201CR___ _________:45 ↔ UND_0201CR___ _________:47
- [Flush]: UND_0201CR___ _________:43 ↔ UND_0201CR___ _________:46
- [Flush]: UND_0201CR___ _________:44 ↔ UND_0201CR___ _________:47
- Flush:734: UND_0201CR___ _________:35 ↔ UND_0201CR___ _________:48
- Flush:735: UND_0201CR___ _________:30 ↔ UND_0201CR___ _________:40
- Flush:736: UND_0201CR___ _________:32 ↔ UND_0201CR___ _________:49
- Flush:737: UND_0201CR___ _________:6 ↔ UND_0201CR___ _________:33
- [Flush]: UND_0201CR___ _________:51 ↔ UND_0201CR___ _________:54
- [Flush]: UND_0201CR___ _________:53 ↔ UND_0201CR___ _________:54
- [Flush]: UND_0201CR___ _________:50 ↔ UND_0201CR___ _________:54
- [Flush]: UND_0201CR___ _________:52 ↔ UND_0201CR___ _________:55
- [Flush]: UND_0201CR___ _________:51 ↔ UND_0201CR___ _________:52
- [Flush]: UND_0201CR___ _________:57 ↔ UND_0201CR___ _________:59
- [Flush]: UND_0201CR___ _________:58 ↔ UND_0201CR___ _________:59
- [Flush]: UND_0201CR___ _________:56 ↔ UND_0201CR___ _________:59
- [Flush]: UND_0201CR___ _________:55 ↔ UND_0201CR___ _________:57
- [Flush]: UND_0201CR___ _________:53 ↔ UND_0201CR___ _________:56
- [Flush]: UND_0201CR___ _________:54 ↔ UND_0201CR___ _________:57
- [Flush]: UND_0201CR___ _________:61 ↔ UND_0201CR___ _________:64
- [Flush]: UND_0201CR___ _________:63 ↔ UND_0201CR___ _________:64
- [Flush]: UND_0201CR___ _________:60 ↔ UND_0201CR___ _________:64
- [Flush]: UND_0201CR___ _________:62 ↔ UND_0201CR___ _________:65
- [Flush]: UND_0201CR___ _________:61 ↔ UND_0201CR___ _________:62
- [Flush]: UND_0201CR___ _________:66 ↔ UND_0201CR___ _________:67
- [Flush]: UND_0201CR___ _________:65 ↔ UND_0201CR___ _________:66
- [Flush]: UND_0201CR___ _________:64 ↔ UND_0201CR___ _________:66
- [Flush]: UND_0201CR___ _________:69 ↔ UND_0201CR___ _________:72
- [Flush]: UND_0201CR___ _________:71 ↔ UND_0201CR___ _________:72
- [Flush]: UND_0201CR___ _________:68 ↔ UND_0201CR___ _________:72
- [Flush]: UND_0201CR___ _________:70 ↔ UND_0201CR___ _________:73
- [Flush]: UND_0201CR___ _________:69 ↔ UND_0201CR___ _________:70
- [Flush]: UND_0201CR___ _________:75 ↔ UND_0201CR___ _________:77
- [Flush]: UND_0201CR___ _________:76 ↔ UND_0201CR___ _________:77
- [Flush]: UND_0201CR___ _________:74 ↔ UND_0201CR___ _________:77
- [Flush]: UND_0201CR___ _________:73 ↔ UND_0201CR___ _________:75
- [Flush]: UND_0201CR___ _________:71 ↔ UND_0201CR___ _________:74
- [Flush]: UND_0201CR___ _________:72 ↔ UND_0201CR___ _________:75
- Flush:768: UND_0201CR___ _________:44 ↔ UND_0201CR___ _________:51
- Flush:769: UND_0201CR___ _________:43 ↔ UND_0201CR___ _________:76
- Flush:770: UND_0201CR___ _________:49 ↔ UND_0201CR___ _________:57
- Flush:771: UND_0201CR___ _________:60 ↔ UND_0201CR___ _________:67
- Flush:772: UND_0201CR___ _________:8 ↔ UND_0201CR___ _________:40
- Flush:773: UND_0201CR___ _________:69 ↔ UND_0201CR___ _________:77
- [Flush]: UND_0201CR___ _________:79 ↔ UND_0201CR___ _________:82
- [Flush]: UND_0201CR___ _________:81 ↔ UND_0201CR___ _________:82
- [Flush]: UND_0201CR___ _________:78 ↔ UND_0201CR___ _________:82
- [Flush]: UND_0201CR___ _________:80 ↔ UND_0201CR___ _________:83
- [Flush]: UND_0201CR___ _________:79 ↔ UND_0201CR___ _________:80
- [Flush]: UND_0201CR___ _________:86 ↔ UND_0201CR___ _________:89
- [Flush]: UND_0201CR___ _________:88 ↔ UND_0201CR___ _________:89
- [Flush]: UND_0201CR___ _________:85 ↔ UND_0201CR___ _________:89
- [Flush]: UND_0201CR___ _________:87 ↔ UND_0201CR___ _________:90
- [Flush]: UND_0201CR___ _________:86 ↔ UND_0201CR___ _________:87
- [Flush]: UND_0201CR___ _________:92 ↔ UND_0201CR___ _________:94
- [Flush]: UND_0201CR___ _________:93 ↔ UND_0201CR___ _________:94
- [Flush]: UND_0201CR___ _________:91 ↔ UND_0201CR___ _________:94
- [Flush]: UND_0201CR___ _________:90 ↔ UND_0201CR___ _________:92
- [Flush]: UND_0201CR___ _________:88 ↔ UND_0201CR___ _________:91